# Autodesk Inventor assembly: _TOP
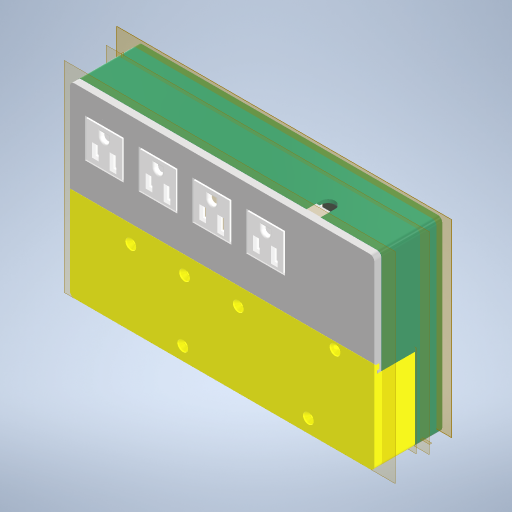
[picture p0: Inventor's stored thumbnail of the model, 512x512]
Saved by Autodesk Inventor 2023.3 (Build 273359000, 359)
## iProperties
Created: 2023-07-31
Part Number: _TOP
Document SubType Name: Assembly
Designer: atrus
Author: atrus
## Documents named in this file (5)
- C:\Users\atrus\Dropbox\elec\Mechanical\ReefVoltEssential\_TOP.iam
- C:\Users\atrus\Dropbox\elec\Mechanical\ReefVoltEssential\ECAD\reefvolt_power_essentials_ESP32.iam
- C:\Users\atrus\Dropbox\elec\Mechanical\ReefVoltEssential\RV_ES_Bottom.ipt
- C:\Users\atrus\Dropbox\elec\Mechanical\ReefVoltEssential\RV_ES_TopHV.ipt
- C:\Users\atrus\Dropbox\elec\Mechanical\ReefVoltEssential\RV_ES_TopLV.ipt
## Components (4 placed, 4 different names)
1. reefvolt_power_essentials_ESP32:2 [sub-assembly] — Angle:1, Mate:1, Mate:2, Mate:3, Mate:8, Mate:10, Flush:3, Flush:4, Flush:5, Flush:6
2. RV_ES_Bottom:1 — Angle:1, Mate:1, Mate:2, Mate:3, Mate:8, Mate:10, Flush:1, Flush:2, Mate:11, Mate:12, Flush:7, Flush:8, Mate:13, Flush:9, Flush:10
3. RV_ES_TopHV:1 — Flush:1, Flush:2, Mate:11, Mate:12, Flush:3, Flush:4, Flush:5, Flush:6
4. RV_ES_TopLV:1 — Flush:7, Flush:8, Mate:13, Flush:9, Flush:10
## Relationships (19: Flush 10, Mate 8, Angle 1)
- Angle:1 (0 deg): reefvolt_power_essentials_ESP32:2 ↔ RV_ES_Bottom:1
- Mate:1 (10 mm): reefvolt_power_essentials_ESP32:2 ↔ RV_ES_Bottom:1
- Mate:2 (-3.81 mm): reefvolt_power_essentials_ESP32:2 ↔ RV_ES_Bottom:1
- Mate:3 (-3.81 mm): reefvolt_power_essentials_ESP32:2 ↔ RV_ES_Bottom:1
- Mate:8: reefvolt_power_essentials_ESP32:2 ↔ RV_ES_Bottom:1
- Mate:10: reefvolt_power_essentials_ESP32:2 ↔ RV_ES_Bottom:1
- Flush:1: RV_ES_Bottom:1 ↔ RV_ES_TopHV:1
- Flush:2: RV_ES_Bottom:1 ↔ RV_ES_TopHV:1
- Mate:11 (0.1 mm): RV_ES_Bottom:1 ↔ RV_ES_TopHV:1
- Mate:12: RV_ES_Bottom:1 ↔ RV_ES_TopHV:1
- Flush:3 (0.2032 mm): reefvolt_power_essentials_ESP32:2 ↔ RV_ES_TopHV:1
- Flush:4 (0.508 mm): reefvolt_power_essentials_ESP32:2 ↔ RV_ES_TopHV:1
- Flush:5 (0.9906 mm): reefvolt_power_essentials_ESP32:2 ↔ RV_ES_TopHV:1
- Flush:6 (0.508 mm): reefvolt_power_essentials_ESP32:2 ↔ RV_ES_TopHV:1
- Flush:7: RV_ES_Bottom:1 ↔ RV_ES_TopLV:1
- Flush:8: RV_ES_Bottom:1 ↔ RV_ES_TopLV:1
- Mate:13 (0.1016 mm): RV_ES_Bottom:1 ↔ RV_ES_TopLV:1
- Flush:9 (0.1016 mm): RV_ES_Bottom:1 ↔ RV_ES_TopLV:1
- Flush:10 (0.1016 mm): RV_ES_Bottom:1 ↔ RV_ES_TopLV:1
